# Autodesk Inventor assembly: chwytak_zlozenie
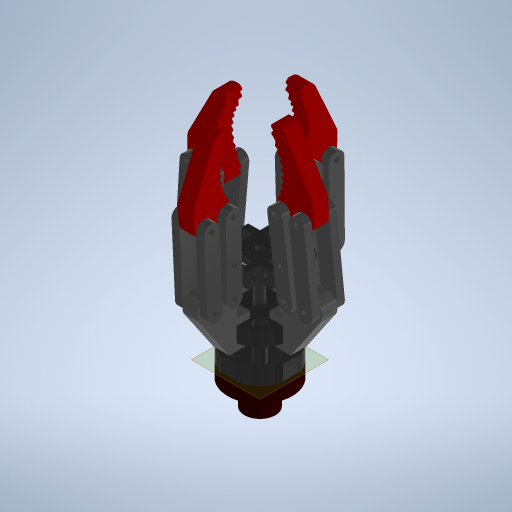
[picture p0: Inventor's stored thumbnail of the model, 512x512]
Saved by Autodesk Inventor 2023 (Build 270158000, 158)
## iProperties
Created: 2023-06-03
Part Number: chwytak_zlozenie
Document SubType Name: Assembly
Designer: komputer
Author: komputer
## Documents named in this file (6)
- C:\Users\Kamil\Desktop\KONARM_2\chwytak\chwytak_zlozenie — kopia.iam
- C:\Users\Kamil\Desktop\KONARM_2\chwytak\chwytak_podstawa.iam
- C:\Users\Kamil\Desktop\KONARM_2\chwytak\palec.iam
- C:\Users\Kamil\Desktop\KONARM_2\chwytak\krzyzyk.iam
- C:\Users\Kamil\Desktop\KONARM_2\chwytak\ShaftToScrewCoupler.ipt
- C:\Users\Kamil\Desktop\KONARM_2\uchwytna wal.ipt
## Components (8 placed, 5 different names)
1. chwytak_podstawa:1 [sub-assembly] — Mate:1, Mate:2, Mate:3, Mate:4, Mate:5, Mate:6, Mate:7, Mate:8, Mate:9, Równoległe:1
2. palec:1 [sub-assembly] — Mate:3, Mate:4
3. palec:2 [sub-assembly] — Mate:5, Mate:6
4. palec:3 [sub-assembly] — Mate:7, Mate:8
5. palec:4 [sub-assembly] — Mate:1, Mate:2
6. krzyzyk:1 [sub-assembly] — Mate:9, Mate:10
7. ShaftToScrewCoupler:1 — Mate:10
8. uchwytna wal:1 — Równoległe:1
## Relationships (11: Mate 10, Flush 1)
- Mate:1 (0.5 mm): chwytak_podstawa:1 ↔ palec:4
- Mate:2: chwytak_podstawa:1 ↔ palec:4
- Mate:3 (0.5 mm): chwytak_podstawa:1 ↔ palec:1
- Mate:4: chwytak_podstawa:1 ↔ palec:1
- Mate:5 (0.5 mm): chwytak_podstawa:1 ↔ palec:2
- Mate:6: chwytak_podstawa:1 ↔ palec:2
- Mate:7 (0.5 mm): chwytak_podstawa:1 ↔ palec:3
- Mate:8: chwytak_podstawa:1 ↔ palec:3
- Mate:9: chwytak_podstawa:1 ↔ krzyzyk:1
- Mate:10: krzyzyk:1 ↔ ShaftToScrewCoupler:1
- Równoległe:1 [Flush]: chwytak_podstawa:1 ↔ uchwytna wal:1
